# Autodesk Inventor assembly: first_floor_simplified
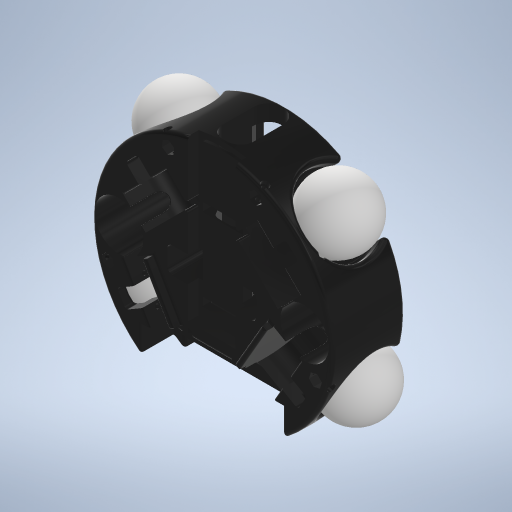
[picture p0: Inventor's stored thumbnail of the model, 512x512]
Saved by Autodesk Inventor 2023 (Build 270158000, 158)
## iProperties
Created: 2022-08-10
Part Number: first_floor_simplified
Document SubType Name: Assembly
Designer: victo
Author: victo
## Documents named in this file (3)
- C:\Users\victo\Documents\MATLAB\CAD\Inventor\first_floor\first_floor_simplified.iam
- C:\Users\victo\Documents\MATLAB\CAD\Inventor\first_floor\Base_RoboCIn_simplified.ipt
- C:\Users\victo\Documents\MATLAB\CAD\Inventor\first_floor\Wheel\wheel_simplified.ipt
## Components (5 placed, 2 different names)
1. Base_RoboCIn_simplified:1 — Coincidente:1, Coincidente:2, Coincidente:3, Coincidente:4
2. wheel_simplified:1 — Coincidente:1
3. wheel_simplified:2 — Coincidente:2
4. wheel_simplified:3 — Coincidente:3
5. wheel_simplified:4 — Coincidente:4
## Relationships (4: Mate 4)
- Coincidente:1 [Mate]: Base_RoboCIn_simplified:1 ↔ wheel_simplified:1
- Coincidente:2 [Mate]: Base_RoboCIn_simplified:1 ↔ wheel_simplified:2
- Coincidente:3 [Mate]: Base_RoboCIn_simplified:1 ↔ wheel_simplified:3
- Coincidente:4 [Mate]: Base_RoboCIn_simplified:1 ↔ wheel_simplified:4
